# Autodesk Inventor assembly: cata
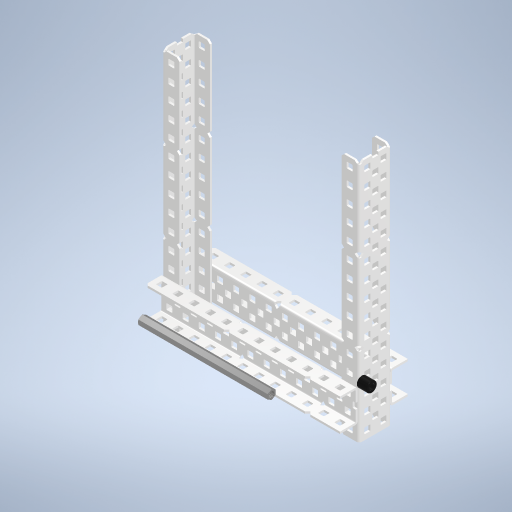
[picture p0: Inventor's stored thumbnail of the model, 512x512]
Saved by Autodesk Inventor 2023 (Build 270158000, 158)
## iProperties
Created: 2023-09-27
Part Number: cata
Document SubType Name: Assembly
Designer: Robodox
Author: Robodox
## Documents named in this file (5)
- C:\Users\Robodox\Documents\GitHub\2023-599Z\BBot-Cad\cata.iam
- C:\Users\Robodox\Documents\GitHub\2023-599Z\BBot-Cad\2020 VRC Library-BNS-SID-YY-EZ\2020 BNS-VRC-SID-YY Library\Structure\C-Channels\2 Wide\Alu C-Chan 2x12.ipt
- C:\Users\Robodox\Documents\GitHub\2023-599Z\BBot-Cad\2020 VRC Library-BNS-SID-YY-EZ\2020 BNS-VRC-SID-YY Library\Structure\C-Channels\2 Wide\Alu C-Chan 2x15.ipt
- C:\Users\Robodox\Documents\GitHub\2023-599Z\BBot-Cad\2020 VRC Library-BNS-SID-YY-EZ\2020 BNS-VRC-SID-YY Library\Structure\Standoffs\Standoff 4.00_.ipt
- C:\Users\Robodox\Documents\GitHub\2023-599Z\BBot-Cad\2020 VRC Library-BNS-SID-YY-EZ\2020 BNS-VRC-SID-YY Library\Motion\Spacers\Spacer (Plastic), 8mm_.ipt
## Components (6 placed, 5 different names)
1. Alu C-Chan 2x15:2 — Mate:1, Mate:2
2. cata bottom bar 2x15:3 — Mate:3, Mate:4, Mate:5
3. Alu C-Chan 2x12:1 — Mate:1, Mate:2, Mate:3, Mate:4
4. Alu C-Chan 2x12:2 — Mate:5
5. Standoff 4.00_:1
6. Spacer (Plastic), 8mm_:1
## Relationships (5: Mate 5)
- Mate:1: Alu C-Chan 2x15:2 ↔ Alu C-Chan 2x12:1
- Mate:2: Alu C-Chan 2x15:2 ↔ Alu C-Chan 2x12:1
- Mate:3: cata bottom bar 2x15:3 ↔ Alu C-Chan 2x12:1
- Mate:4: cata bottom bar 2x15:3 ↔ Alu C-Chan 2x12:1
- Mate:5: cata bottom bar 2x15:3 ↔ Alu C-Chan 2x12:2
